# Autodesk Inventor assembly: Кронштейн
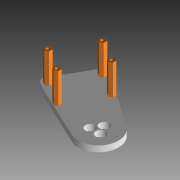
[picture p0: Inventor's stored thumbnail of the model, 180x180]
Saved by Autodesk Inventor 2022 (Build 260153000, 153)
## iProperties
Created: 2025-01-23
Part Number: Кронштейн
Document SubType Name: Assembly
Designer: Ivan
Mass: 24.7676 g
Surface Area: 133.939 cm^2
Volume: 24.7676 cm^3
Density: 1 g/cm^3
Author: Ivan
Title: Кронштейн
## Documents named in this file (3)
- E:\Предпроф 2025\Shoter_1_ZIP\Кронштейн.iam
- E:\Предпроф 2025\Shoter_1_ZIP\Кронштейн_разлив.ipt
- E:\Предпроф 2025\Shoter_1_ZIP\Стойка м3х40.ipt
## Components (5 placed, 2 different names)
1. Кронштейн_разлив:1 — Совмещение:1, Совмещение:2, Совмещение:3, Совмещение:4, Совмещение:5, Совмещение:6, Совмещение:7, Совмещение:8
2. Стойка м3х40:1 — Совмещение:4, Совмещение:6
3. Стойка м3х40:2 — Совмещение:2, Совмещение:8
4. Стойка м3х40:3 — Совмещение:1, Совмещение:7
5. Стойка м3х40:4 — Совмещение:3, Совмещение:5
## Relationships (8: Mate 8)
- Совмещение:1 [Mate]: Кронштейн_разлив:1 ↔ Стойка м3х40:3
- Совмещение:2 [Mate]: Кронштейн_разлив:1 ↔ Стойка м3х40:2
- Совмещение:3 [Mate]: Кронштейн_разлив:1 ↔ Стойка м3х40:4
- Совмещение:4 [Mate]: Кронштейн_разлив:1 ↔ Стойка м3х40:1
- Совмещение:5 [Mate]: Кронштейн_разлив:1 ↔ Стойка м3х40:4
- Совмещение:6 [Mate]: Кронштейн_разлив:1 ↔ Стойка м3х40:1
- Совмещение:7 [Mate]: Кронштейн_разлив:1 ↔ Стойка м3х40:3
- Совмещение:8 [Mate]: Кронштейн_разлив:1 ↔ Стойка м3х40:2
